# Autodesk Inventor assembly: daeyoung_profile
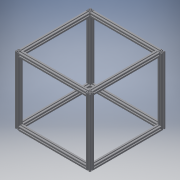
[picture p0: Inventor's stored thumbnail of the model, 180x180]
Saved by Autodesk Inventor 2016 (Build 200138000, 138)
## iProperties
Created: 2024-05-31
Part Number: daeyoung_profile
Material: 일반
Document SubType Name: Assembly
Designer: pc
Author: pc
## Documents named in this file (2)
- D:\CAD_HCH\240531\대영프로파일\daeyoung_profile.iam
- D:\CAD_HCH\240531\대영프로파일\daeyoung_profile.ipt
## Components (12 placed, 1 different names)
1. daeyoung_profile:1 — 메이트:1, 메이트:3, 메이트:4, 메이트:5
2. daeyoung_profile:2 — 메이트:1, 메이트:2
3. daeyoung_profile:3 — 메이트:3
4. daeyoung_profile:4 — 메이트:5
5. daeyoung_profile:5 — 메이트:4, 메이트:6
6. daeyoung_profile:6 — 메이트:7, 메이트:10
7. daeyoung_profile:7 — 메이트:2, 메이트:7, 메이트:11
8. daeyoung_profile:8 — 메이트:9, 메이트:10
9. daeyoung_profile:9 — 메이트:8, 메이트:9
10. daeyoung_profile:10 — 메이트:11
11. daeyoung_profile:11 — 메이트:6, 메이트:8, 메이트:12
12. daeyoung_profile:12 — 메이트:12
## Relationships (12: Mate 12)
- 메이트:1 [Mate]: daeyoung_profile:1 ↔ daeyoung_profile:2
- 메이트:2 [Mate]: daeyoung_profile:2 ↔ daeyoung_profile:7
- 메이트:3 [Mate]: daeyoung_profile:1 ↔ daeyoung_profile:3
- 메이트:4 [Mate]: daeyoung_profile:1 ↔ daeyoung_profile:5
- 메이트:5 [Mate]: daeyoung_profile:1 ↔ daeyoung_profile:4
- 메이트:6 [Mate]: daeyoung_profile:5 ↔ daeyoung_profile:11
- 메이트:7 [Mate]: daeyoung_profile:6 ↔ daeyoung_profile:7
- 메이트:8 [Mate]: daeyoung_profile:9 ↔ daeyoung_profile:11
- 메이트:9 [Mate]: daeyoung_profile:8 ↔ daeyoung_profile:9
- 메이트:10 [Mate]: daeyoung_profile:6 ↔ daeyoung_profile:8
- 메이트:11 [Mate]: daeyoung_profile:7 ↔ daeyoung_profile:10
- 메이트:12 [Mate]: daeyoung_profile:11 ↔ daeyoung_profile:12
